# Autodesk Inventor assembly: cycloid_top_bottom_assy
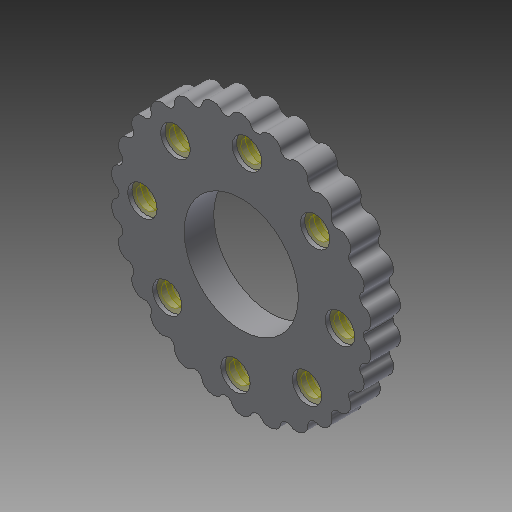
[picture p0: Inventor's stored thumbnail of the model, 512x512]
Saved by Autodesk Inventor 2019.3 (Build 233278000, 278)
## iProperties
Created: 2019-08-28
Part Number: cycloid_top_bottom_assy
Document SubType Name: Assembly
Designer: cdi
Author: cdi
## Documents named in this file (3)
- C:\Users\cdi\SynologyDrive\workspace_inventor\2019_06_19.MT4008_actuator\cycloid_gear_design_v1\cycloid_top_bottom_assy.iam
- C:\Users\cdi\SynologyDrive\workspace_inventor\2019_06_19.MT4008_actuator\cycloid_gear_design_v1\cycloid_top_bottom.ipt
- C:\Users\cdi\SynologyDrive\workspace_inventor\2019_06_19.MT4008_actuator\cycloid_gear_design_v1\bearing_8x5x2.5.ipt
## Components (17 placed, 2 different names)
1. cycloid_top_bottom:1 — Mate:1, Mate:2, Mate:3
2. bearing_8x5x2.5:1 — Mate:1, Mate:2, Mate:4
3. bearing_8x5x2.5:2 — Mate:3, Mate:4
4. bearing_8x5x2.5:3
5. bearing_8x5x2.5:4
6. bearing_8x5x2.5:5
7. bearing_8x5x2.5:6
8. bearing_8x5x2.5:7
9. bearing_8x5x2.5:8
10. bearing_8x5x2.5:9
11. bearing_8x5x2.5:10
12. bearing_8x5x2.5:11
13. bearing_8x5x2.5:12
14. bearing_8x5x2.5:13
15. bearing_8x5x2.5:14
16. bearing_8x5x2.5:15
17. bearing_8x5x2.5:16
## Component patterns: (8 elements, first: bearing_8x5x2.5:1 + bearing_8x5x2.5:2)
## Relationships (4: Mate 4)
- Mate:1: cycloid_top_bottom:1 ↔ bearing_8x5x2.5:1
- Mate:2: cycloid_top_bottom:1 ↔ bearing_8x5x2.5:1
- Mate:3: cycloid_top_bottom:1 ↔ bearing_8x5x2.5:2
- Mate:4: bearing_8x5x2.5:1 ↔ bearing_8x5x2.5:2
